# Autodesk Inventor assembly: 3U_sq_tube_amsat
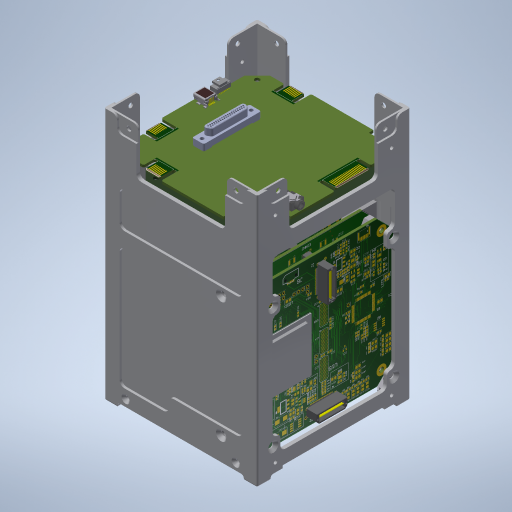
[picture p0: Inventor's stored thumbnail of the model, 512x512]
Saved by Autodesk Inventor 2023 (Build 270158000, 158)
## iProperties
Created: 2018-08-12
Part Number: 3U_sq_tube_amsat
Document SubType Name: Assembly
Designer: RDavis
Author: RDavis
## iProperties of the stored document MemberDocs/xAaaaqbcaAaaaaaaaAaaaqxjcCb
Created: 2018-08-12
Part Number: 3U_sq_tube_amsat
Document SubType Name: Assembly
Designer: RDavis
Author: RDavis
## Documents named in this file (8)
- E:\Dropbox\AMSAT\CAD_backup_frequent_files_20200629\3U_sq_tube_amsat.iam
- E:\Dropbox\AMSAT\CAD_backup_frequent_files_20200629\3U_sq_tube_amsat.ipt
- E:\Dropbox\AMSAT\CAD_backup_frequent_files_20200629\E310.iam
- E:\Dropbox\AMSAT\CAD_backup_frequent_files_20200629\pcb_stack_tall.iam
- E:\Dropbox\AMSAT\CAD_backup_frequent_files_20200629\pcb_stack_short.iam
- E:\Dropbox\AMSAT\CAD_backup_frequent_files_20200629\PCB_IU.iam
- E:\Dropbox\AMSAT\CAD_backup_frequent_files_20200629\nub_minusZ_switch.iam
- E:\Dropbox\AMSAT\CAD_backup_frequent_files_20200629\nub_minusZ_1.ipt
## Components (9 placed, 7 different names)
1. 3U_sq_tube_amsat:1 — Flush:1, Flush:2, Flush:3, Mate:1, Flush:4, Flush:20, Flush:5, Flush:11, Flush:18, Mate:17, Mate:18, Flush:19, Mate:19, Mate:20, Flush:22, Mate:23, Mate:24, Flush:23, Mate:25, Mate:26
2. E310:1 [sub-assembly] — Mate:1, Mate:15, Flush:4
3. pcb_stack_tall:1 [sub-assembly] — Flush:20, Flush:5, Mate:22
4. pcb_stack_short:1 [sub-assembly] — Mate:12, Mate:10, Flush:21
5. PCB_IU:1 [sub-assembly] — Flush:11, Mate:13, Flush:12, Mate:10, Flush:21
6. nub_minusZ_switch:1 [sub-assembly] — Flush:18, Mate:17, Mate:18
7. nub_minusZ_switch:2 [sub-assembly] — Flush:19, Mate:19, Mate:20
8. nub_minusZ_1:1 — Flush:22, Mate:23, Mate:24
9. nub_minusZ_1:2 — Flush:23, Mate:25, Mate:26
## Relationships (27: Mate 14, Flush 13)
- Flush:1: 3U_sq_tube_amsat:1
- Flush:2: 3U_sq_tube_amsat:1
- Flush:3: 3U_sq_tube_amsat:1
- Mate:1 (3 mm): 3U_sq_tube_amsat:1 ↔ E310:1
- Mate:15: E310:1
- Flush:4 (7 mm): 3U_sq_tube_amsat:1 ↔ E310:1
- Flush:20 (8.15 mm): 3U_sq_tube_amsat:1 ↔ pcb_stack_tall:1
- Flush:5 (10 mm): 3U_sq_tube_amsat:1 ↔ pcb_stack_tall:1
- Mate:22: pcb_stack_tall:1
- Mate:12: pcb_stack_short:1
- Mate:10 (8.15 mm): pcb_stack_short:1 ↔ PCB_IU:1
- Flush:11 (140 mm): 3U_sq_tube_amsat:1 ↔ PCB_IU:1
- Mate:13: PCB_IU:1
- Flush:12: PCB_IU:1
- Flush:18: 3U_sq_tube_amsat:1 ↔ nub_minusZ_switch:1
- Mate:17: 3U_sq_tube_amsat:1 ↔ nub_minusZ_switch:1
- Mate:18: 3U_sq_tube_amsat:1 ↔ nub_minusZ_switch:1
- Flush:19: 3U_sq_tube_amsat:1 ↔ nub_minusZ_switch:2
- Mate:19: 3U_sq_tube_amsat:1 ↔ nub_minusZ_switch:2
- Mate:20: 3U_sq_tube_amsat:1 ↔ nub_minusZ_switch:2
- Flush:21 (1.5 mm): pcb_stack_short:1 ↔ PCB_IU:1
- Flush:22: 3U_sq_tube_amsat:1 ↔ nub_minusZ_1:1
- Mate:23: 3U_sq_tube_amsat:1 ↔ nub_minusZ_1:1
- Mate:24: 3U_sq_tube_amsat:1 ↔ nub_minusZ_1:1
- Flush:23: 3U_sq_tube_amsat:1 ↔ nub_minusZ_1:2
- Mate:25: 3U_sq_tube_amsat:1 ↔ nub_minusZ_1:2
- Mate:26: 3U_sq_tube_amsat:1 ↔ nub_minusZ_1:2
